# Autodesk Inventor assembly: SCST6-8
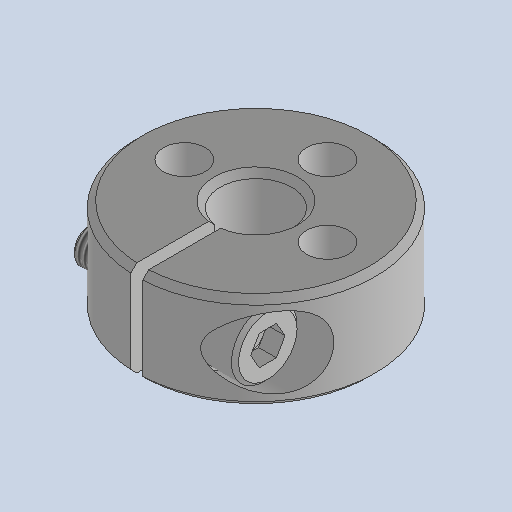
[picture p0: Inventor's stored thumbnail of the model, 512x512]
Saved by Autodesk Inventor 2024 (Build 280153000, 153)
## iProperties
Category: PARTsolutions
Company: MISUMI
Created: 2025-08-19
Part Number: SCST6-8
Catalog Web Link: www.cadenas.de
Description: SCST, PSCST, SSCST, SCSTR, PSCSTR, SSCSTR-Set Collars - Slit 3 Hole/3 Tap - Standard Type -
Vendor: MISUMI
Document SubType Name: Assembly
Designer: psAdmin
Manufacturer: MISUMI
Mass: 1.9526 g
Surface Area: 18.0804 cm^2
Volume: 1.9526 cm^3
Density: 1 g/cm^3
PSOL_IDENT_0: {$CADENAS_DATA/23d-libs/misumi/metric/03_set_collars/scst_asmtab.prj},218 {VTYP=3D},{STYP=ASSTAB},{N
PSOL_IDENT_1: B=SCST6-8},{LINA=SCST6-8},{NN=SCST, PSCST, SSCST, SCSTR, PSCSTR, SSCSTR},{DATE=29.11.2024 04:05:21},
PSOL_IDENT_2: {GEOMDATE=15.09.2021 06:07:55},{VERSION=},{LINEID=220},{WBVAR=TS,MAT,ST,BS},{WBNUMERIC=BS}  {NB=SCST
PSOL_IDENT_3: 6-8},{LINA=SCST6-8},{KT=DUMMY},{PN=SCST6-8},{TYPE=SCST},{TS=3H},{TSALG= '3H' , '3-Hole' , '3T' , '3-
PSOL_IDENT_4: Tapped' },{MAT=S45C},{ST=BO},{STALG= 'BO' , 'Black Oxide' , 'ENP' , 'Electroless Nickel Plating' },{
PSOL_IDENT_5: AC=Hex Socket Head Cap Screw 1 pc.},{ACMAT=4137 Alloy Steel},{D=6},{BS=8},{BALG= 8 , 10 },{D1=20},{M=
PSOL_IDENT_6: M3},{M3D=3},{DD=3.4},{R=3.00},{W=1.0},{X=6.0},{Y=4},{P=12},{C=0.5},{S=3.5},{M1=-},{M13D=0},{L=12},{P
PSOL_IDENT_7: PATH=scst/scst_templ.prj}
NB: SCST6-8
NN: SCST, PSCST, SSCST, SCSTR, PSCSTR, SSCSTR
NT: Set Collars - Slit 3 Hole/3 Tap - Standard Type -
NBSYN: $PN.
LINA: SCST6-8
CATALOG: Misumi
PN: SCST6-8
TS: 3-Hole
MAT: 1045 Carbon Steel
ST: Black Oxide
AC: Hex Socket Head Cap Screw 1 pc.
ACMAT: 4137 Alloy Steel
D: 6
BS: 8
D1: 20
M: M3
DD: 3.4
R: 3
W: 1
X: 6
Y: 4
P: 12
C: 0.5
S: 3.5
M1: -
SUPPLIER: MISUMI
ARTICLENO: SCST6-8
BOMINFO: SCST6-8
CREATOR: CADENAS GmbH
Title: SCST6-8
Author: Cadenas PARTsolutions
Comments: Set Collars - Slit 3 Hole/3 Tap - Standard Type -
## Documents named in this file (3)
- C:\Users\HosodaLab2\OneDrive - Kyoto University\ドキュメント\Inventor\arm2\SCST6-8.iam
- C:\Users\HosodaLab2\OneDrive - Kyoto University\ドキュメント\Inventor\arm2\SCST6-8b.ipt
- C:\Users\HosodaLab2\OneDrive - Kyoto University\ドキュメント\Inventor\arm2\BOLT3-12.ipt
## Components (2 placed, 2 different names)
1. SCST6-8b:1 — to_bolt_XY@1 <-> to_cp_XY@2, to_bolt_Z@1 <-> to_cp_Z@2, to_bolt_YZ@1 <-> to_cp_YZ@2
2. BOLT3-12:1 — to_bolt_XY@1 <-> to_cp_XY@2, to_bolt_Z@1 <-> to_cp_Z@2, to_bolt_YZ@1 <-> to_cp_YZ@2
## Relationships (3: Mate 2, Angle 1)
- to_bolt_XY@1 <-> to_cp_XY@2 [Mate]: SCST6-8b:1 ↔ BOLT3-12:1
- to_bolt_Z@1 <-> to_cp_Z@2 [Mate]: SCST6-8b:1 ↔ BOLT3-12:1
- to_bolt_YZ@1 <-> to_cp_YZ@2 [Angle] (0 deg): SCST6-8b:1 ↔ BOLT3-12:1
